# Autodesk Inventor assembly: Ball End
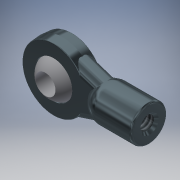
[picture p0: Inventor's stored thumbnail of the model, 180x180]
Saved by Autodesk Inventor 2019 (Build 230136000, 136)
## iProperties
Created: 2019-12-01
Part Number: Ball End
Document SubType Name: Assembly
Designer: Jopa
Author: Jopa
## Documents named in this file (3)
- C:\Users\Jopa\Desktop\Suspension\Ball End.iam
- C:\Users\Jopa\Desktop\Suspension\Ball End.ipt
- C:\Users\Jopa\Desktop\Suspension\0.25 Ball.ipt
## Components (2 placed, 2 different names)
1. Ball End:1 — Mate:1, Mate:2
2. 0.25 Ball:1 — Mate:1, Mate:2
## Relationships (2: Mate 2)
- Mate:1: Ball End:1 ↔ 0.25 Ball:1
- Mate:2: Ball End:1 ↔ 0.25 Ball:1
